(part 1 of 2)
# Autodesk Inventor assembly: Pins
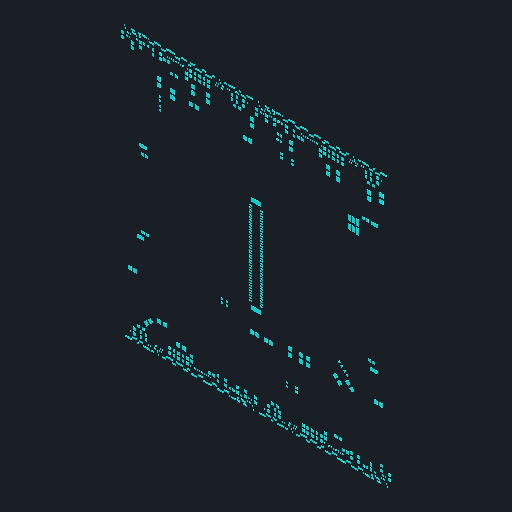
[picture p0: Inventor's stored thumbnail of the model, 512x512]
Saved by Autodesk Inventor 2027 (Build 310192060, 192F)
## iProperties
Created: 2026-07-14
Part Number: Pins
Description: PART--DESC
Document SubType Name: Assembly
Designer: caleb
Author: caleb
Revision Number: NONE
## Documents named in this file (559)
- C:\Users\caleb\Desktop\Shared\Software\Hardware\ETL\modules\Tamale v2.0\module_r50\Pins.iam
- C:\Users\caleb\Desktop\Shared\Software\Hardware\ETL\modules\Tamale v2.0\module_r50\1.ipt
- C:\Users\caleb\Desktop\Shared\Software\Hardware\ETL\modules\Tamale v2.0\module_r50\1_1.ipt
- C:\Users\caleb\Desktop\Shared\Software\Hardware\ETL\modules\Tamale v2.0\module_r50\1_2.ipt
- C:\Users\caleb\Desktop\Shared\Software\Hardware\ETL\modules\Tamale v2.0\module_r50\1_3.ipt
- C:\Users\caleb\Desktop\Shared\Software\Hardware\ETL\modules\Tamale v2.0\module_r50\1_4.ipt
- C:\Users\caleb\Desktop\Shared\Software\Hardware\ETL\modules\Tamale v2.0\module_r50\1_5.ipt
- C:\Users\caleb\Desktop\Shared\Software\Hardware\ETL\modules\Tamale v2.0\module_r50\1_6.ipt
- C:\Users\caleb\Desktop\Shared\Software\Hardware\ETL\modules\Tamale v2.0\module_r50\1_7.ipt
- C:\Users\caleb\Desktop\Shared\Software\Hardware\ETL\modules\Tamale v2.0\module_r50\1_8.ipt
- C:\Users\caleb\Desktop\Shared\Software\Hardware\ETL\modules\Tamale v2.0\module_r50\1_9.ipt
- C:\Users\caleb\Desktop\Shared\Software\Hardware\ETL\modules\Tamale v2.0\module_r50\1_10.ipt
- C:\Users\caleb\Desktop\Shared\Software\Hardware\ETL\modules\Tamale v2.0\module_r50\1_11.ipt
- C:\Users\caleb\Desktop\Shared\Software\Hardware\ETL\modules\Tamale v2.0\module_r50\1_12.ipt
- C:\Users\caleb\Desktop\Shared\Software\Hardware\ETL\modules\Tamale v2.0\module_r50\1_13.ipt
- C:\Users\caleb\Desktop\Shared\Software\Hardware\ETL\modules\Tamale v2.0\module_r50\1_14.ipt
- C:\Users\caleb\Desktop\Shared\Software\Hardware\ETL\modules\Tamale v2.0\module_r50\1_15.ipt
- C:\Users\caleb\Desktop\Shared\Software\Hardware\ETL\modules\Tamale v2.0\module_r50\1_16.ipt
- C:\Users\caleb\Desktop\Shared\Software\Hardware\ETL\modules\Tamale v2.0\module_r50\1_17.ipt
- C:\Users\caleb\Desktop\Shared\Software\Hardware\ETL\modules\Tamale v2.0\module_r50\1_18.ipt
- C:\Users\caleb\Desktop\Shared\Software\Hardware\ETL\modules\Tamale v2.0\module_r50\1_19.ipt
- C:\Users\caleb\Desktop\Shared\Software\Hardware\ETL\modules\Tamale v2.0\module_r50\1_20.ipt
- C:\Users\caleb\Desktop\Shared\Software\Hardware\ETL\modules\Tamale v2.0\module_r50\1_21.ipt
- C:\Users\caleb\Desktop\Shared\Software\Hardware\ETL\modules\Tamale v2.0\module_r50\1_22.ipt
- C:\Users\caleb\Desktop\Shared\Software\Hardware\ETL\modules\Tamale v2.0\module_r50\1_23.ipt
- C:\Users\caleb\Desktop\Shared\Software\Hardware\ETL\modules\Tamale v2.0\module_r50\1_24.ipt
- C:\Users\caleb\Desktop\Shared\Software\Hardware\ETL\modules\Tamale v2.0\module_r50\1_25.ipt
- C:\Users\caleb\Desktop\Shared\Software\Hardware\ETL\modules\Tamale v2.0\module_r50\1_26.ipt
- C:\Users\caleb\Desktop\Shared\Software\Hardware\ETL\modules\Tamale v2.0\module_r50\1_27.ipt
- C:\Users\caleb\Desktop\Shared\Software\Hardware\ETL\modules\Tamale v2.0\module_r50\1_28.ipt
- C:\Users\caleb\Desktop\Shared\Software\Hardware\ETL\modules\Tamale v2.0\module_r50\1_29.ipt
- C:\Users\caleb\Desktop\Shared\Software\Hardware\ETL\modules\Tamale v2.0\module_r50\1_30.ipt
- C:\Users\caleb\Desktop\Shared\Software\Hardware\ETL\modules\Tamale v2.0\module_r50\1_31.ipt
- C:\Users\caleb\Desktop\Shared\Software\Hardware\ETL\modules\Tamale v2.0\module_r50\1_32.ipt
- C:\Users\caleb\Desktop\Shared\Software\Hardware\ETL\modules\Tamale v2.0\module_r50\1_33.ipt
- C:\Users\caleb\Desktop\Shared\Software\Hardware\ETL\modules\Tamale v2.0\module_r50\1_34.ipt
- C:\Users\caleb\Desktop\Shared\Software\Hardware\ETL\modules\Tamale v2.0\module_r50\1_35.ipt
- C:\Users\caleb\Desktop\Shared\Software\Hardware\ETL\modules\Tamale v2.0\module_r50\1_36.ipt
- C:\Users\caleb\Desktop\Shared\Software\Hardware\ETL\modules\Tamale v2.0\module_r50\1_37.ipt
- C:\Users\caleb\Desktop\Shared\Software\Hardware\ETL\modules\Tamale v2.0\module_r50\1_38.ipt
- C:\Users\caleb\Desktop\Shared\Software\Hardware\ETL\modules\Tamale v2.0\module_r50\1_39.ipt
- C:\Users\caleb\Desktop\Shared\Software\Hardware\ETL\modules\Tamale v2.0\module_r50\1_40.ipt
- C:\Users\caleb\Desktop\Shared\Software\Hardware\ETL\modules\Tamale v2.0\module_r50\1_41.ipt
- C:\Users\caleb\Desktop\Shared\Software\Hardware\ETL\modules\Tamale v2.0\module_r50\1_42.ipt
- C:\Users\caleb\Desktop\Shared\Software\Hardware\ETL\modules\Tamale v2.0\module_r50\1_43.ipt
- C:\Users\caleb\Desktop\Shared\Software\Hardware\ETL\modules\Tamale v2.0\module_r50\1_44.ipt
- C:\Users\caleb\Desktop\Shared\Software\Hardware\ETL\modules\Tamale v2.0\module_r50\1_45.ipt
- C:\Users\caleb\Desktop\Shared\Software\Hardware\ETL\modules\Tamale v2.0\module_r50\1_46.ipt
- C:\Users\caleb\Desktop\Shared\Software\Hardware\ETL\modules\Tamale v2.0\module_r50\1_47.ipt
- C:\Users\caleb\Desktop\Shared\Software\Hardware\ETL\modules\Tamale v2.0\module_r50\1_48.ipt
- C:\Users\caleb\Desktop\Shared\Software\Hardware\ETL\modules\Tamale v2.0\module_r50\1_49.ipt
- C:\Users\caleb\Desktop\Shared\Software\Hardware\ETL\modules\Tamale v2.0\module_r50\1_50.ipt
- C:\Users\caleb\Desktop\Shared\Software\Hardware\ETL\modules\Tamale v2.0\module_r50\1_51.ipt
- C:\Users\caleb\Desktop\Shared\Software\Hardware\ETL\modules\Tamale v2.0\module_r50\1_52.ipt
- C:\Users\caleb\Desktop\Shared\Software\Hardware\ETL\modules\Tamale v2.0\module_r50\1_53.ipt
- C:\Users\caleb\Desktop\Shared\Software\Hardware\ETL\modules\Tamale v2.0\module_r50\1_54.ipt
- C:\Users\caleb\Desktop\Shared\Software\Hardware\ETL\modules\Tamale v2.0\module_r50\1_55.ipt
- C:\Users\caleb\Desktop\Shared\Software\Hardware\ETL\modules\Tamale v2.0\module_r50\1_56.ipt
- C:\Users\caleb\Desktop\Shared\Software\Hardware\ETL\modules\Tamale v2.0\module_r50\1_57.ipt
- C:\Users\caleb\Desktop\Shared\Software\Hardware\ETL\modules\Tamale v2.0\module_r50\1_58.ipt
- C:\Users\caleb\Desktop\Shared\Software\Hardware\ETL\modules\Tamale v2.0\module_r50\1_59.ipt
- C:\Users\caleb\Desktop\Shared\Software\Hardware\ETL\modules\Tamale v2.0\module_r50\1_60.ipt
- C:\Users\caleb\Desktop\Shared\Software\Hardware\ETL\modules\Tamale v2.0\module_r50\1_61.ipt
- C:\Users\caleb\Desktop\Shared\Software\Hardware\ETL\modules\Tamale v2.0\module_r50\1_62.ipt
- C:\Users\caleb\Desktop\Shared\Software\Hardware\ETL\modules\Tamale v2.0\module_r50\1_63.ipt
- C:\Users\caleb\Desktop\Shared\Software\Hardware\ETL\modules\Tamale v2.0\module_r50\1_64.ipt
- C:\Users\caleb\Desktop\Shared\Software\Hardware\ETL\modules\Tamale v2.0\module_r50\1_65.ipt
- C:\Users\caleb\Desktop\Shared\Software\Hardware\ETL\modules\Tamale v2.0\module_r50\1_66.ipt
- C:\Users\caleb\Desktop\Shared\Software\Hardware\ETL\modules\Tamale v2.0\module_r50\1_67.ipt
- C:\Users\caleb\Desktop\Shared\Software\Hardware\ETL\modules\Tamale v2.0\module_r50\1_68.ipt
- C:\Users\caleb\Desktop\Shared\Software\Hardware\ETL\modules\Tamale v2.0\module_r50\1_69.ipt
- C:\Users\caleb\Desktop\Shared\Software\Hardware\ETL\modules\Tamale v2.0\module_r50\1_70.ipt
- C:\Users\caleb\Desktop\Shared\Software\Hardware\ETL\modules\Tamale v2.0\module_r50\1_71.ipt
- C:\Users\caleb\Desktop\Shared\Software\Hardware\ETL\modules\Tamale v2.0\module_r50\1_72.ipt
- C:\Users\caleb\Desktop\Shared\Software\Hardware\ETL\modules\Tamale v2.0\module_r50\1_73.ipt
- C:\Users\caleb\Desktop\Shared\Software\Hardware\ETL\modules\Tamale v2.0\module_r50\1_74.ipt
- C:\Users\caleb\Desktop\Shared\Software\Hardware\ETL\modules\Tamale v2.0\module_r50\1_75.ipt
- C:\Users\caleb\Desktop\Shared\Software\Hardware\ETL\modules\Tamale v2.0\module_r50\1_76.ipt
- C:\Users\caleb\Desktop\Shared\Software\Hardware\ETL\modules\Tamale v2.0\module_r50\1_77.ipt
- C:\Users\caleb\Desktop\Shared\Software\Hardware\ETL\modules\Tamale v2.0\module_r50\1_78.ipt
- C:\Users\caleb\Desktop\Shared\Software\Hardware\ETL\modules\Tamale v2.0\module_r50\1_79.ipt
- C:\Users\caleb\Desktop\Shared\Software\Hardware\ETL\modules\Tamale v2.0\module_r50\1_80.ipt
- C:\Users\caleb\Desktop\Shared\Software\Hardware\ETL\modules\Tamale v2.0\module_r50\1_81.ipt
- C:\Users\caleb\Desktop\Shared\Software\Hardware\ETL\modules\Tamale v2.0\module_r50\1_82.ipt
- C:\Users\caleb\Desktop\Shared\Software\Hardware\ETL\modules\Tamale v2.0\module_r50\1_83.ipt
- C:\Users\caleb\Desktop\Shared\Software\Hardware\ETL\modules\Tamale v2.0\module_r50\1_84.ipt
- C:\Users\caleb\Desktop\Shared\Software\Hardware\ETL\modules\Tamale v2.0\module_r50\1_85.ipt
- C:\Users\caleb\Desktop\Shared\Software\Hardware\ETL\modules\Tamale v2.0\module_r50\1_86.ipt
- C:\Users\caleb\Desktop\Shared\Software\Hardware\ETL\modules\Tamale v2.0\module_r50\1_87.ipt
- C:\Users\caleb\Desktop\Shared\Software\Hardware\ETL\modules\Tamale v2.0\module_r50\1_88.ipt
- C:\Users\caleb\Desktop\Shared\Software\Hardware\ETL\modules\Tamale v2.0\module_r50\1_89.ipt
- C:\Users\caleb\Desktop\Shared\Software\Hardware\ETL\modules\Tamale v2.0\module_r50\1_90.ipt
- C:\Users\caleb\Desktop\Shared\Software\Hardware\ETL\modules\Tamale v2.0\module_r50\1_91.ipt
- C:\Users\caleb\Desktop\Shared\Software\Hardware\ETL\modules\Tamale v2.0\module_r50\1_92.ipt
- C:\Users\caleb\Desktop\Shared\Software\Hardware\ETL\modules\Tamale v2.0\module_r50\1_93.ipt
- C:\Users\caleb\Desktop\Shared\Software\Hardware\ETL\modules\Tamale v2.0\module_r50\1_94.ipt
- C:\Users\caleb\Desktop\Shared\Software\Hardware\ETL\modules\Tamale v2.0\module_r50\1_95.ipt
- C:\Users\caleb\Desktop\Shared\Software\Hardware\ETL\modules\Tamale v2.0\module_r50\1_96.ipt
- C:\Users\caleb\Desktop\Shared\Software\Hardware\ETL\modules\Tamale v2.0\module_r50\1_97.ipt
- C:\Users\caleb\Desktop\Shared\Software\Hardware\ETL\modules\Tamale v2.0\module_r50\1_98.ipt
- C:\Users\caleb\Desktop\Shared\Software\Hardware\ETL\modules\Tamale v2.0\module_r50\1_99.ipt
- C:\Users\caleb\Desktop\Shared\Software\Hardware\ETL\modules\Tamale v2.0\module_r50\1_100.ipt
- C:\Users\caleb\Desktop\Shared\Software\Hardware\ETL\modules\Tamale v2.0\module_r50\1_101.ipt
- C:\Users\caleb\Desktop\Shared\Software\Hardware\ETL\modules\Tamale v2.0\module_r50\1_102.ipt
- C:\Users\caleb\Desktop\Shared\Software\Hardware\ETL\modules\Tamale v2.0\module_r50\1_103.ipt
- C:\Users\caleb\Desktop\Shared\Software\Hardware\ETL\modules\Tamale v2.0\module_r50\1_104.ipt
- C:\Users\caleb\Desktop\Shared\Software\Hardware\ETL\modules\Tamale v2.0\module_r50\1_105.ipt
- C:\Users\caleb\Desktop\Shared\Software\Hardware\ETL\modules\Tamale v2.0\module_r50\1_106.ipt
- C:\Users\caleb\Desktop\Shared\Software\Hardware\ETL\modules\Tamale v2.0\module_r50\1_107.ipt
- C:\Users\caleb\Desktop\Shared\Software\Hardware\ETL\modules\Tamale v2.0\module_r50\1_108.ipt
- C:\Users\caleb\Desktop\Shared\Software\Hardware\ETL\modules\Tamale v2.0\module_r50\1_109.ipt
- C:\Users\caleb\Desktop\Shared\Software\Hardware\ETL\modules\Tamale v2.0\module_r50\1_110.ipt
- C:\Users\caleb\Desktop\Shared\Software\Hardware\ETL\modules\Tamale v2.0\module_r50\1_111.ipt
- C:\Users\caleb\Desktop\Shared\Software\Hardware\ETL\modules\Tamale v2.0\module_r50\1_112.ipt
- C:\Users\caleb\Desktop\Shared\Software\Hardware\ETL\modules\Tamale v2.0\module_r50\10.ipt
- C:\Users\caleb\Desktop\Shared\Software\Hardware\ETL\modules\Tamale v2.0\module_r50\11.ipt
- C:\Users\caleb\Desktop\Shared\Software\Hardware\ETL\modules\Tamale v2.0\module_r50\12.ipt
- C:\Users\caleb\Desktop\Shared\Software\Hardware\ETL\modules\Tamale v2.0\module_r50\13.ipt
- C:\Users\caleb\Desktop\Shared\Software\Hardware\ETL\modules\Tamale v2.0\module_r50\14.ipt
- C:\Users\caleb\Desktop\Shared\Software\Hardware\ETL\modules\Tamale v2.0\module_r50\15.ipt
- C:\Users\caleb\Desktop\Shared\Software\Hardware\ETL\modules\Tamale v2.0\module_r50\16.ipt
- C:\Users\caleb\Desktop\Shared\Software\Hardware\ETL\modules\Tamale v2.0\module_r50\17.ipt
- C:\Users\caleb\Desktop\Shared\Software\Hardware\ETL\modules\Tamale v2.0\module_r50\18.ipt
- C:\Users\caleb\Desktop\Shared\Software\Hardware\ETL\modules\Tamale v2.0\module_r50\19.ipt
- C:\Users\caleb\Desktop\Shared\Software\Hardware\ETL\modules\Tamale v2.0\module_r50\2.ipt
- C:\Users\caleb\Desktop\Shared\Software\Hardware\ETL\modules\Tamale v2.0\module_r50\2_1.ipt
- C:\Users\caleb\Desktop\Shared\Software\Hardware\ETL\modules\Tamale v2.0\module_r50\2_2.ipt
- C:\Users\caleb\Desktop\Shared\Software\Hardware\ETL\modules\Tamale v2.0\module_r50\2_3.ipt
- C:\Users\caleb\Desktop\Shared\Software\Hardware\ETL\modules\Tamale v2.0\module_r50\2_4.ipt
- C:\Users\caleb\Desktop\Shared\Software\Hardware\ETL\modules\Tamale v2.0\module_r50\2_5.ipt
- C:\Users\caleb\Desktop\Shared\Software\Hardware\ETL\modules\Tamale v2.0\module_r50\2_6.ipt
- C:\Users\caleb\Desktop\Shared\Software\Hardware\ETL\modules\Tamale v2.0\module_r50\2_7.ipt
- C:\Users\caleb\Desktop\Shared\Software\Hardware\ETL\modules\Tamale v2.0\module_r50\2_8.ipt
- C:\Users\caleb\Desktop\Shared\Software\Hardware\ETL\modules\Tamale v2.0\module_r50\2_9.ipt
- C:\Users\caleb\Desktop\Shared\Software\Hardware\ETL\modules\Tamale v2.0\module_r50\2_10.ipt
- C:\Users\caleb\Desktop\Shared\Software\Hardware\ETL\modules\Tamale v2.0\module_r50\2_11.ipt
- C:\Users\caleb\Desktop\Shared\Software\Hardware\ETL\modules\Tamale v2.0\module_r50\2_12.ipt
- C:\Users\caleb\Desktop\Shared\Software\Hardware\ETL\modules\Tamale v2.0\module_r50\2_13.ipt
- C:\Users\caleb\Desktop\Shared\Software\Hardware\ETL\modules\Tamale v2.0\module_r50\2_14.ipt
- C:\Users\caleb\Desktop\Shared\Software\Hardware\ETL\modules\Tamale v2.0\module_r50\2_15.ipt
- C:\Users\caleb\Desktop\Shared\Software\Hardware\ETL\modules\Tamale v2.0\module_r50\2_16.ipt
- C:\Users\caleb\Desktop\Shared\Software\Hardware\ETL\modules\Tamale v2.0\module_r50\2_17.ipt
- C:\Users\caleb\Desktop\Shared\Software\Hardware\ETL\modules\Tamale v2.0\module_r50\2_18.ipt
- C:\Users\caleb\Desktop\Shared\Software\Hardware\ETL\modules\Tamale v2.0\module_r50\2_19.ipt
- C:\Users\caleb\Desktop\Shared\Software\Hardware\ETL\modules\Tamale v2.0\module_r50\2_20.ipt
- C:\Users\caleb\Desktop\Shared\Software\Hardware\ETL\modules\Tamale v2.0\module_r50\2_21.ipt
- C:\Users\caleb\Desktop\Shared\Software\Hardware\ETL\modules\Tamale v2.0\module_r50\2_22.ipt
- C:\Users\caleb\Desktop\Shared\Software\Hardware\ETL\modules\Tamale v2.0\module_r50\2_23.ipt
- C:\Users\caleb\Desktop\Shared\Software\Hardware\ETL\modules\Tamale v2.0\module_r50\2_24.ipt
- C:\Users\caleb\Desktop\Shared\Software\Hardware\ETL\modules\Tamale v2.0\module_r50\2_25.ipt
- C:\Users\caleb\Desktop\Shared\Software\Hardware\ETL\modules\Tamale v2.0\module_r50\2_26.ipt
- C:\Users\caleb\Desktop\Shared\Software\Hardware\ETL\modules\Tamale v2.0\module_r50\2_27.ipt
- C:\Users\caleb\Desktop\Shared\Software\Hardware\ETL\modules\Tamale v2.0\module_r50\2_28.ipt
- C:\Users\caleb\Desktop\Shared\Software\Hardware\ETL\modules\Tamale v2.0\module_r50\2_29.ipt
- C:\Users\caleb\Desktop\Shared\Software\Hardware\ETL\modules\Tamale v2.0\module_r50\2_30.ipt
- C:\Users\caleb\Desktop\Shared\Software\Hardware\ETL\modules\Tamale v2.0\module_r50\2_31.ipt
- C:\Users\caleb\Desktop\Shared\Software\Hardware\ETL\modules\Tamale v2.0\module_r50\2_32.ipt
- C:\Users\caleb\Desktop\Shared\Software\Hardware\ETL\modules\Tamale v2.0\module_r50\2_33.ipt
- C:\Users\caleb\Desktop\Shared\Software\Hardware\ETL\modules\Tamale v2.0\module_r50\2_34.ipt
- C:\Users\caleb\Desktop\Shared\Software\Hardware\ETL\modules\Tamale v2.0\module_r50\2_35.ipt
- C:\Users\caleb\Desktop\Shared\Software\Hardware\ETL\modules\Tamale v2.0\module_r50\2_36.ipt
- C:\Users\caleb\Desktop\Shared\Software\Hardware\ETL\modules\Tamale v2.0\module_r50\2_37.ipt
- C:\Users\caleb\Desktop\Shared\Software\Hardware\ETL\modules\Tamale v2.0\module_r50\2_38.ipt
- C:\Users\caleb\Desktop\Shared\Software\Hardware\ETL\modules\Tamale v2.0\module_r50\2_39.ipt
- C:\Users\caleb\Desktop\Shared\Software\Hardware\ETL\modules\Tamale v2.0\module_r50\2_40.ipt
- C:\Users\caleb\Desktop\Shared\Software\Hardware\ETL\modules\Tamale v2.0\module_r50\2_41.ipt
- C:\Users\caleb\Desktop\Shared\Software\Hardware\ETL\modules\Tamale v2.0\module_r50\2_42.ipt
- C:\Users\caleb\Desktop\Shared\Software\Hardware\ETL\modules\Tamale v2.0\module_r50\2_43.ipt
- C:\Users\caleb\Desktop\Shared\Software\Hardware\ETL\modules\Tamale v2.0\module_r50\2_44.ipt
- C:\Users\caleb\Desktop\Shared\Software\Hardware\ETL\modules\Tamale v2.0\module_r50\2_45.ipt
- C:\Users\caleb\Desktop\Shared\Software\Hardware\ETL\modules\Tamale v2.0\module_r50\2_46.ipt
- C:\Users\caleb\Desktop\Shared\Software\Hardware\ETL\modules\Tamale v2.0\module_r50\2_47.ipt
- C:\Users\caleb\Desktop\Shared\Software\Hardware\ETL\modules\Tamale v2.0\module_r50\2_48.ipt
- C:\Users\caleb\Desktop\Shared\Software\Hardware\ETL\modules\Tamale v2.0\module_r50\2_49.ipt
- C:\Users\caleb\Desktop\Shared\Software\Hardware\ETL\modules\Tamale v2.0\module_r50\2_50.ipt
- C:\Users\caleb\Desktop\Shared\Software\Hardware\ETL\modules\Tamale v2.0\module_r50\2_51.ipt
- C:\Users\caleb\Desktop\Shared\Software\Hardware\ETL\modules\Tamale v2.0\module_r50\2_52.ipt
- C:\Users\caleb\Desktop\Shared\Software\Hardware\ETL\modules\Tamale v2.0\module_r50\2_53.ipt
- C:\Users\caleb\Desktop\Shared\Software\Hardware\ETL\modules\Tamale v2.0\module_r50\2_54.ipt
- C:\Users\caleb\Desktop\Shared\Software\Hardware\ETL\modules\Tamale v2.0\module_r50\2_55.ipt
- C:\Users\caleb\Desktop\Shared\Software\Hardware\ETL\modules\Tamale v2.0\module_r50\2_56.ipt
- C:\Users\caleb\Desktop\Shared\Software\Hardware\ETL\modules\Tamale v2.0\module_r50\2_57.ipt
- C:\Users\caleb\Desktop\Shared\Software\Hardware\ETL\modules\Tamale v2.0\module_r50\2_58.ipt
- C:\Users\caleb\Desktop\Shared\Software\Hardware\ETL\modules\Tamale v2.0\module_r50\2_59.ipt
- C:\Users\caleb\Desktop\Shared\Software\Hardware\ETL\modules\Tamale v2.0\module_r50\2_60.ipt
- C:\Users\caleb\Desktop\Shared\Software\Hardware\ETL\modules\Tamale v2.0\module_r50\2_61.ipt
- C:\Users\caleb\Desktop\Shared\Software\Hardware\ETL\modules\Tamale v2.0\module_r50\2_62.ipt
- C:\Users\caleb\Desktop\Shared\Software\Hardware\ETL\modules\Tamale v2.0\module_r50\2_63.ipt
- C:\Users\caleb\Desktop\Shared\Software\Hardware\ETL\modules\Tamale v2.0\module_r50\2_64.ipt
- C:\Users\caleb\Desktop\Shared\Software\Hardware\ETL\modules\Tamale v2.0\module_r50\2_65.ipt
- C:\Users\caleb\Desktop\Shared\Software\Hardware\ETL\modules\Tamale v2.0\module_r50\2_66.ipt
- C:\Users\caleb\Desktop\Shared\Software\Hardware\ETL\modules\Tamale v2.0\module_r50\2_67.ipt
- C:\Users\caleb\Desktop\Shared\Software\Hardware\ETL\modules\Tamale v2.0\module_r50\2_68.ipt
- C:\Users\caleb\Desktop\Shared\Software\Hardware\ETL\modules\Tamale v2.0\module_r50\2_69.ipt
- C:\Users\caleb\Desktop\Shared\Software\Hardware\ETL\modules\Tamale v2.0\module_r50\2_70.ipt
- C:\Users\caleb\Desktop\Shared\Software\Hardware\ETL\modules\Tamale v2.0\module_r50\2_71.ipt
- C:\Users\caleb\Desktop\Shared\Software\Hardware\ETL\modules\Tamale v2.0\module_r50\2_72.ipt
- C:\Users\caleb\Desktop\Shared\Software\Hardware\ETL\modules\Tamale v2.0\module_r50\2_73.ipt
- C:\Users\caleb\Desktop\Shared\Software\Hardware\ETL\modules\Tamale v2.0\module_r50\2_74.ipt
- C:\Users\caleb\Desktop\Shared\Software\Hardware\ETL\modules\Tamale v2.0\module_r50\2_75.ipt
- C:\Users\caleb\Desktop\Shared\Software\Hardware\ETL\modules\Tamale v2.0\module_r50\2_76.ipt
- C:\Users\caleb\Desktop\Shared\Software\Hardware\ETL\modules\Tamale v2.0\module_r50\2_77.ipt
- C:\Users\caleb\Desktop\Shared\Software\Hardware\ETL\modules\Tamale v2.0\module_r50\2_78.ipt
- C:\Users\caleb\Desktop\Shared\Software\Hardware\ETL\modules\Tamale v2.0\module_r50\2_79.ipt
- C:\Users\caleb\Desktop\Shared\Software\Hardware\ETL\modules\Tamale v2.0\module_r50\2_80.ipt
- C:\Users\caleb\Desktop\Shared\Software\Hardware\ETL\modules\Tamale v2.0\module_r50\2_81.ipt
- C:\Users\caleb\Desktop\Shared\Software\Hardware\ETL\modules\Tamale v2.0\module_r50\2_82.ipt
- C:\Users\caleb\Desktop\Shared\Software\Hardware\ETL\modules\Tamale v2.0\module_r50\2_83.ipt
- C:\Users\caleb\Desktop\Shared\Software\Hardware\ETL\modules\Tamale v2.0\module_r50\2_84.ipt
- C:\Users\caleb\Desktop\Shared\Software\Hardware\ETL\modules\Tamale v2.0\module_r50\2_85.ipt
- C:\Users\caleb\Desktop\Shared\Software\Hardware\ETL\modules\Tamale v2.0\module_r50\2_86.ipt
- C:\Users\caleb\Desktop\Shared\Software\Hardware\ETL\modules\Tamale v2.0\module_r50\2_87.ipt
- C:\Users\caleb\Desktop\Shared\Software\Hardware\ETL\modules\Tamale v2.0\module_r50\2_88.ipt
- C:\Users\caleb\Desktop\Shared\Software\Hardware\ETL\modules\Tamale v2.0\module_r50\2_89.ipt
- C:\Users\caleb\Desktop\Shared\Software\Hardware\ETL\modules\Tamale v2.0\module_r50\2_90.ipt
- C:\Users\caleb\Desktop\Shared\Software\Hardware\ETL\modules\Tamale v2.0\module_r50\2_91.ipt
- C:\Users\caleb\Desktop\Shared\Software\Hardware\ETL\modules\Tamale v2.0\module_r50\2_92.ipt
- C:\Users\caleb\Desktop\Shared\Software\Hardware\ETL\modules\Tamale v2.0\module_r50\2_93.ipt
- C:\Users\caleb\Desktop\Shared\Software\Hardware\ETL\modules\Tamale v2.0\module_r50\2_94.ipt
- C:\Users\caleb\Desktop\Shared\Software\Hardware\ETL\modules\Tamale v2.0\module_r50\2_95.ipt
- C:\Users\caleb\Desktop\Shared\Software\Hardware\ETL\modules\Tamale v2.0\module_r50\2_96.ipt
- C:\Users\caleb\Desktop\Shared\Software\Hardware\ETL\modules\Tamale v2.0\module_r50\2_97.ipt
- C:\Users\caleb\Desktop\Shared\Software\Hardware\ETL\modules\Tamale v2.0\module_r50\2_98.ipt
- C:\Users\caleb\Desktop\Shared\Software\Hardware\ETL\modules\Tamale v2.0\module_r50\2_99.ipt
- C:\Users\caleb\Desktop\Shared\Software\Hardware\ETL\modules\Tamale v2.0\module_r50\2_100.ipt
- C:\Users\caleb\Desktop\Shared\Software\Hardware\ETL\modules\Tamale v2.0\module_r50\2_101.ipt
- C:\Users\caleb\Desktop\Shared\Software\Hardware\ETL\modules\Tamale v2.0\module_r50\2_102.ipt
- C:\Users\caleb\Desktop\Shared\Software\Hardware\ETL\modules\Tamale v2.0\module_r50\2_103.ipt
- C:\Users\caleb\Desktop\Shared\Software\Hardware\ETL\modules\Tamale v2.0\module_r50\2_104.ipt
- C:\Users\caleb\Desktop\Shared\Software\Hardware\ETL\modules\Tamale v2.0\module_r50\2_105.ipt
- C:\Users\caleb\Desktop\Shared\Software\Hardware\ETL\modules\Tamale v2.0\module_r50\2_106.ipt
- C:\Users\caleb\Desktop\Shared\Software\Hardware\ETL\modules\Tamale v2.0\module_r50\2_107.ipt
- C:\Users\caleb\Desktop\Shared\Software\Hardware\ETL\modules\Tamale v2.0\module_r50\2_108.ipt
- C:\Users\caleb\Desktop\Shared\Software\Hardware\ETL\modules\Tamale v2.0\module_r50\2_109.ipt
- C:\Users\caleb\Desktop\Shared\Software\Hardware\ETL\modules\Tamale v2.0\module_r50\2_110.ipt
- C:\Users\caleb\Desktop\Shared\Software\Hardware\ETL\modules\Tamale v2.0\module_r50\2_111.ipt
- C:\Users\caleb\Desktop\Shared\Software\Hardware\ETL\modules\Tamale v2.0\module_r50\2_112.ipt
- C:\Users\caleb\Desktop\Shared\Software\Hardware\ETL\modules\Tamale v2.0\module_r50\20.ipt
- C:\Users\caleb\Desktop\Shared\Software\Hardware\ETL\modules\Tamale v2.0\module_r50\21.ipt
- C:\Users\caleb\Desktop\Shared\Software\Hardware\ETL\modules\Tamale v2.0\module_r50\22.ipt
- C:\Users\caleb\Desktop\Shared\Software\Hardware\ETL\modules\Tamale v2.0\module_r50\23.ipt
- C:\Users\caleb\Desktop\Shared\Software\Hardware\ETL\modules\Tamale v2.0\module_r50\24.ipt
- C:\Users\caleb\Desktop\Shared\Software\Hardware\ETL\modules\Tamale v2.0\module_r50\25.ipt
- C:\Users\caleb\Desktop\Shared\Software\Hardware\ETL\modules\Tamale v2.0\module_r50\26.ipt
- C:\Users\caleb\Desktop\Shared\Software\Hardware\ETL\modules\Tamale v2.0\module_r50\27.ipt
- C:\Users\caleb\Desktop\Shared\Software\Hardware\ETL\modules\Tamale v2.0\module_r50\28.ipt
- C:\Users\caleb\Desktop\Shared\Software\Hardware\ETL\modules\Tamale v2.0\module_r50\29.ipt
- C:\Users\caleb\Desktop\Shared\Software\Hardware\ETL\modules\Tamale v2.0\module_r50\3.ipt
- C:\Users\caleb\Desktop\Shared\Software\Hardware\ETL\modules\Tamale v2.0\module_r50\3_1.ipt
- C:\Users\caleb\Desktop\Shared\Software\Hardware\ETL\modules\Tamale v2.0\module_r50\3_2.ipt
- C:\Users\caleb\Desktop\Shared\Software\Hardware\ETL\modules\Tamale v2.0\module_r50\30.ipt
- C:\Users\caleb\Desktop\Shared\Software\Hardware\ETL\modules\Tamale v2.0\module_r50\31.ipt
- C:\Users\caleb\Desktop\Shared\Software\Hardware\ETL\modules\Tamale v2.0\module_r50\32.ipt
- C:\Users\caleb\Desktop\Shared\Software\Hardware\ETL\modules\Tamale v2.0\module_r50\33.ipt
- C:\Users\caleb\Desktop\Shared\Software\Hardware\ETL\modules\Tamale v2.0\module_r50\34.ipt
- C:\Users\caleb\Desktop\Shared\Software\Hardware\ETL\modules\Tamale v2.0\module_r50\35.ipt
- C:\Users\caleb\Desktop\Shared\Software\Hardware\ETL\modules\Tamale v2.0\module_r50\36.ipt
- C:\Users\caleb\Desktop\Shared\Software\Hardware\ETL\modules\Tamale v2.0\module_r50\37.ipt
- C:\Users\caleb\Desktop\Shared\Software\Hardware\ETL\modules\Tamale v2.0\module_r50\38.ipt
- C:\Users\caleb\Desktop\Shared\Software\Hardware\ETL\modules\Tamale v2.0\module_r50\39.ipt
- C:\Users\caleb\Desktop\Shared\Software\Hardware\ETL\modules\Tamale v2.0\module_r50\4.ipt
- C:\Users\caleb\Desktop\Shared\Software\Hardware\ETL\modules\Tamale v2.0\module_r50\40.ipt
- C:\Users\caleb\Desktop\Shared\Software\Hardware\ETL\modules\Tamale v2.0\module_r50\41.ipt
- C:\Users\caleb\Desktop\Shared\Software\Hardware\ETL\modules\Tamale v2.0\module_r50\42.ipt
- C:\Users\caleb\Desktop\Shared\Software\Hardware\ETL\modules\Tamale v2.0\module_r50\43.ipt
- C:\Users\caleb\Desktop\Shared\Software\Hardware\ETL\modules\Tamale v2.0\module_r50\44.ipt
- C:\Users\caleb\Desktop\Shared\Software\Hardware\ETL\modules\Tamale v2.0\module_r50\45.ipt
- C:\Users\caleb\Desktop\Shared\Software\Hardware\ETL\modules\Tamale v2.0\module_r50\46.ipt
- C:\Users\caleb\Desktop\Shared\Software\Hardware\ETL\modules\Tamale v2.0\module_r50\47.ipt
- C:\Users\caleb\Desktop\Shared\Software\Hardware\ETL\modules\Tamale v2.0\module_r50\48.ipt
- C:\Users\caleb\Desktop\Shared\Software\Hardware\ETL\modules\Tamale v2.0\module_r50\49.ipt
- C:\Users\caleb\Desktop\Shared\Software\Hardware\ETL\modules\Tamale v2.0\module_r50\5.ipt
- C:\Users\caleb\Desktop\Shared\Software\Hardware\ETL\modules\Tamale v2.0\module_r50\50.ipt
- C:\Users\caleb\Desktop\Shared\Software\Hardware\ETL\modules\Tamale v2.0\module_r50\51.ipt
- C:\Users\caleb\Desktop\Shared\Software\Hardware\ETL\modules\Tamale v2.0\module_r50\52.ipt
- C:\Users\caleb\Desktop\Shared\Software\Hardware\ETL\modules\Tamale v2.0\module_r50\53.ipt
- C:\Users\caleb\Desktop\Shared\Software\Hardware\ETL\modules\Tamale v2.0\module_r50\54.ipt
- C:\Users\caleb\Desktop\Shared\Software\Hardware\ETL\modules\Tamale v2.0\module_r50\55.ipt
- C:\Users\caleb\Desktop\Shared\Software\Hardware\ETL\modules\Tamale v2.0\module_r50\56.ipt
- C:\Users\caleb\Desktop\Shared\Software\Hardware\ETL\modules\Tamale v2.0\module_r50\57.ipt
- C:\Users\caleb\Desktop\Shared\Software\Hardware\ETL\modules\Tamale v2.0\module_r50\58.ipt
- C:\Users\caleb\Desktop\Shared\Software\Hardware\ETL\modules\Tamale v2.0\module_r50\59.ipt
- C:\Users\caleb\Desktop\Shared\Software\Hardware\ETL\modules\Tamale v2.0\module_r50\6.ipt
- C:\Users\caleb\Desktop\Shared\Software\Hardware\ETL\modules\Tamale v2.0\module_r50\60.ipt
- C:\Users\caleb\Desktop\Shared\Software\Hardware\ETL\modules\Tamale v2.0\module_r50\61.ipt
- C:\Users\caleb\Desktop\Shared\Software\Hardware\ETL\modules\Tamale v2.0\module_r50\62.ipt
- C:\Users\caleb\Desktop\Shared\Software\Hardware\ETL\modules\Tamale v2.0\module_r50\63.ipt
- C:\Users\caleb\Desktop\Shared\Software\Hardware\ETL\modules\Tamale v2.0\module_r50\64.ipt
- C:\Users\caleb\Desktop\Shared\Software\Hardware\ETL\modules\Tamale v2.0\module_r50\65.ipt
- C:\Users\caleb\Desktop\Shared\Software\Hardware\ETL\modules\Tamale v2.0\module_r50\66.ipt
- C:\Users\caleb\Desktop\Shared\Software\Hardware\ETL\modules\Tamale v2.0\module_r50\67.ipt
- C:\Users\caleb\Desktop\Shared\Software\Hardware\ETL\modules\Tamale v2.0\module_r50\68.ipt
- C:\Users\caleb\Desktop\Shared\Software\Hardware\ETL\modules\Tamale v2.0\module_r50\69.ipt
- C:\Users\caleb\Desktop\Shared\Software\Hardware\ETL\modules\Tamale v2.0\module_r50\7.ipt
- C:\Users\caleb\Desktop\Shared\Software\Hardware\ETL\modules\Tamale v2.0\module_r50\70.ipt
- C:\Users\caleb\Desktop\Shared\Software\Hardware\ETL\modules\Tamale v2.0\module_r50\71.ipt
- C:\Users\caleb\Desktop\Shared\Software\Hardware\ETL\modules\Tamale v2.0\module_r50\72.ipt
- C:\Users\caleb\Desktop\Shared\Software\Hardware\ETL\modules\Tamale v2.0\module_r50\73.ipt
- C:\Users\caleb\Desktop\Shared\Software\Hardware\ETL\modules\Tamale v2.0\module_r50\74.ipt
- C:\Users\caleb\Desktop\Shared\Software\Hardware\ETL\modules\Tamale v2.0\module_r50\75.ipt
- C:\Users\caleb\Desktop\Shared\Software\Hardware\ETL\modules\Tamale v2.0\module_r50\76.ipt
- C:\Users\caleb\Desktop\Shared\Software\Hardware\ETL\modules\Tamale v2.0\module_r50\77.ipt
- C:\Users\caleb\Desktop\Shared\Software\Hardware\ETL\modules\Tamale v2.0\module_r50\78.ipt
- C:\Users\caleb\Desktop\Shared\Software\Hardware\ETL\modules\Tamale v2.0\module_r50\8.ipt
- C:\Users\caleb\Desktop\Shared\Software\Hardware\ETL\modules\Tamale v2.0\module_r50\9.ipt
- C:\Users\caleb\Desktop\Shared\Software\Hardware\ETL\modules\Tamale v2.0\module_r50\CLK1280_N.ipt
- C:\Users\caleb\Desktop\Shared\Software\Hardware\ETL\modules\Tamale v2.0\module_r50\CLK1280_N_1.ipt
- C:\Users\caleb\Desktop\Shared\Software\Hardware\ETL\modules\Tamale v2.0\module_r50\CLK1280_N_2.ipt
- C:\Users\caleb\Desktop\Shared\Software\Hardware\ETL\modules\Tamale v2.0\module_r50\CLK1280_N_3.ipt
- C:\Users\caleb\Desktop\Shared\Software\Hardware\ETL\modules\Tamale v2.0\module_r50\CLK1280_P.ipt
- C:\Users\caleb\Desktop\Shared\Software\Hardware\ETL\modules\Tamale v2.0\module_r50\CLK1280_P_1.ipt
- C:\Users\caleb\Desktop\Shared\Software\Hardware\ETL\modules\Tamale v2.0\module_r50\CLK1280_P_2.ipt
- C:\Users\caleb\Desktop\Shared\Software\Hardware\ETL\modules\Tamale v2.0\module_r50\CLK1280_P_3.ipt
- C:\Users\caleb\Desktop\Shared\Software\Hardware\ETL\modules\Tamale v2.0\module_r50\CLK40_N.ipt
- C:\Users\caleb\Desktop\Shared\Software\Hardware\ETL\modules\Tamale v2.0\module_r50\CLK40_N_1.ipt
- C:\Users\caleb\Desktop\Shared\Software\Hardware\ETL\modules\Tamale v2.0\module_r50\CLK40_N_2.ipt
- C:\Users\caleb\Desktop\Shared\Software\Hardware\ETL\modules\Tamale v2.0\module_r50\CLK40_N_3.ipt
- C:\Users\caleb\Desktop\Shared\Software\Hardware\ETL\modules\Tamale v2.0\module_r50\CLK40_P.ipt
- C:\Users\caleb\Desktop\Shared\Software\Hardware\ETL\modules\Tamale v2.0\module_r50\CLK40_P_1.ipt
- C:\Users\caleb\Desktop\Shared\Software\Hardware\ETL\modules\Tamale v2.0\module_r50\CLK40_P_2.ipt
- C:\Users\caleb\Desktop\Shared\Software\Hardware\ETL\modules\Tamale v2.0\module_r50\CLK40_P_3.ipt
- C:\Users\caleb\Desktop\Shared\Software\Hardware\ETL\modules\Tamale v2.0\module_r50\DOL_N.ipt
- C:\Users\caleb\Desktop\Shared\Software\Hardware\ETL\modules\Tamale v2.0\module_r50\DOL_N_1.ipt
- C:\Users\caleb\Desktop\Shared\Software\Hardware\ETL\modules\Tamale v2.0\module_r50\DOL_N_2.ipt
- C:\Users\caleb\Desktop\Shared\Software\Hardware\ETL\modules\Tamale v2.0\module_r50\DOL_N_3.ipt
- C:\Users\caleb\Desktop\Shared\Software\Hardware\ETL\modules\Tamale v2.0\module_r50\DOL_P.ipt
- C:\Users\caleb\Desktop\Shared\Software\Hardware\ETL\modules\Tamale v2.0\module_r50\DOL_P_1.ipt
- C:\Users\caleb\Desktop\Shared\Software\Hardware\ETL\modules\Tamale v2.0\module_r50\DOL_P_2.ipt
- C:\Users\caleb\Desktop\Shared\Software\Hardware\ETL\modules\Tamale v2.0\module_r50\DOL_P_3.ipt
- C:\Users\caleb\Desktop\Shared\Software\Hardware\ETL\modules\Tamale v2.0\module_r50\DOR_N.ipt
- C:\Users\caleb\Desktop\Shared\Software\Hardware\ETL\modules\Tamale v2.0\module_r50\DOR_N_1.ipt
- C:\Users\caleb\Desktop\Shared\Software\Hardware\ETL\modules\Tamale v2.0\module_r50\DOR_N_2.ipt
- C:\Users\caleb\Desktop\Shared\Software\Hardware\ETL\modules\Tamale v2.0\module_r50\DOR_N_3.ipt
- C:\Users\caleb\Desktop\Shared\Software\Hardware\ETL\modules\Tamale v2.0\module_r50\DOR_P.ipt
- C:\Users\caleb\Desktop\Shared\Software\Hardware\ETL\modules\Tamale v2.0\module_r50\DOR_P_1.ipt
- C:\Users\caleb\Desktop\Shared\Software\Hardware\ETL\modules\Tamale v2.0\module_r50\DOR_P_2.ipt
- C:\Users\caleb\Desktop\Shared\Software\Hardware\ETL\modules\Tamale v2.0\module_r50\DOR_P_3.ipt
- C:\Users\caleb\Desktop\Shared\Software\Hardware\ETL\modules\Tamale v2.0\module_r50\FCN.ipt
- C:\Users\caleb\Desktop\Shared\Software\Hardware\ETL\modules\Tamale v2.0\module_r50\FCN_1.ipt
- C:\Users\caleb\Desktop\Shared\Software\Hardware\ETL\modules\Tamale v2.0\module_r50\FCN_2.ipt
- C:\Users\caleb\Desktop\Shared\Software\Hardware\ETL\modules\Tamale v2.0\module_r50\FCN_3.ipt
- C:\Users\caleb\Desktop\Shared\Software\Hardware\ETL\modules\Tamale v2.0\module_r50\FCP.ipt
- C:\Users\caleb\Desktop\Shared\Software\Hardware\ETL\modules\Tamale v2.0\module_r50\FCP_1.ipt
- C:\Users\caleb\Desktop\Shared\Software\Hardware\ETL\modules\Tamale v2.0\module_r50\FCP_2.ipt
- C:\Users\caleb\Desktop\Shared\Software\Hardware\ETL\modules\Tamale v2.0\module_r50\FCP_3.ipt
- C:\Users\caleb\Desktop\Shared\Software\Hardware\ETL\modules\Tamale v2.0\module_r50\I2C_ADDR0.ipt
- C:\Users\caleb\Desktop\Shared\Software\Hardware\ETL\modules\Tamale v2.0\module_r50\I2C_ADDR0_1.ipt
- C:\Users\caleb\Desktop\Shared\Software\Hardware\ETL\modules\Tamale v2.0\module_r50\I2C_ADDR0_2.ipt
- C:\Users\caleb\Desktop\Shared\Software\Hardware\ETL\modules\Tamale v2.0\module_r50\I2C_ADDR0_3.ipt
- C:\Users\caleb\Desktop\Shared\Software\Hardware\ETL\modules\Tamale v2.0\module_r50\I2C_ADDR1.ipt
- C:\Users\caleb\Desktop\Shared\Software\Hardware\ETL\modules\Tamale v2.0\module_r50\I2C_ADDR1_1.ipt
- C:\Users\caleb\Desktop\Shared\Software\Hardware\ETL\modules\Tamale v2.0\module_r50\I2C_ADDR1_2.ipt
- C:\Users\caleb\Desktop\Shared\Software\Hardware\ETL\modules\Tamale v2.0\module_r50\I2C_ADDR1_3.ipt
- C:\Users\caleb\Desktop\Shared\Software\Hardware\ETL\modules\Tamale v2.0\module_r50\I2C_ADDR2.ipt
- C:\Users\caleb\Desktop\Shared\Software\Hardware\ETL\modules\Tamale v2.0\module_r50\I2C_ADDR2_1.ipt
- C:\Users\caleb\Desktop\Shared\Software\Hardware\ETL\modules\Tamale v2.0\module_r50\I2C_ADDR2_2.ipt
- C:\Users\caleb\Desktop\Shared\Software\Hardware\ETL\modules\Tamale v2.0\module_r50\I2C_ADDR2_3.ipt
- C:\Users\caleb\Desktop\Shared\Software\Hardware\ETL\modules\Tamale v2.0\module_r50\I2C_ADDR3.ipt
- C:\Users\caleb\Desktop\Shared\Software\Hardware\ETL\modules\Tamale v2.0\module_r50\I2C_ADDR3_1.ipt
- C:\Users\caleb\Desktop\Shared\Software\Hardware\ETL\modules\Tamale v2.0\module_r50\I2C_ADDR3_2.ipt
- C:\Users\caleb\Desktop\Shared\Software\Hardware\ETL\modules\Tamale v2.0\module_r50\I2C_ADDR3_3.ipt
- C:\Users\caleb\Desktop\Shared\Software\Hardware\ETL\modules\Tamale v2.0\module_r50\I2C_ADDR4.ipt
- C:\Users\caleb\Desktop\Shared\Software\Hardware\ETL\modules\Tamale v2.0\module_r50\I2C_ADDR4_1.ipt
- C:\Users\caleb\Desktop\Shared\Software\Hardware\ETL\modules\Tamale v2.0\module_r50\I2C_ADDR4_2.ipt
- C:\Users\caleb\Desktop\Shared\Software\Hardware\ETL\modules\Tamale v2.0\module_r50\I2C_ADDR4_3.ipt
- C:\Users\caleb\Desktop\Shared\Software\Hardware\ETL\modules\Tamale v2.0\module_r50\POWER1.ipt
- C:\Users\caleb\Desktop\Shared\Software\Hardware\ETL\modules\Tamale v2.0\module_r50\POWER2.ipt
- C:\Users\caleb\Desktop\Shared\Software\Hardware\ETL\modules\Tamale v2.0\module_r50\RSTN.ipt
- C:\Users\caleb\Desktop\Shared\Software\Hardware\ETL\modules\Tamale v2.0\module_r50\RSTN_1.ipt
- C:\Users\caleb\Desktop\Shared\Software\Hardware\ETL\modules\Tamale v2.0\module_r50\RSTN_2.ipt
- C:\Users\caleb\Desktop\Shared\Software\Hardware\ETL\modules\Tamale v2.0\module_r50\RSTN_3.ipt
- C:\Users\caleb\Desktop\Shared\Software\Hardware\ETL\modules\Tamale v2.0\module_r50\SCL.ipt
- C:\Users\caleb\Desktop\Shared\Software\Hardware\ETL\modules\Tamale v2.0\module_r50\SCL_1.ipt
- C:\Users\caleb\Desktop\Shared\Software\Hardware\ETL\modules\Tamale v2.0\module_r50\SCL_2.ipt
- C:\Users\caleb\Desktop\Shared\Software\Hardware\ETL\modules\Tamale v2.0\module_r50\SCL_3.ipt
- C:\Users\caleb\Desktop\Shared\Software\Hardware\ETL\modules\Tamale v2.0\module_r50\SDA.ipt
- C:\Users\caleb\Desktop\Shared\Software\Hardware\ETL\modules\Tamale v2.0\module_r50\SDA_1.ipt
- C:\Users\caleb\Desktop\Shared\Software\Hardware\ETL\modules\Tamale v2.0\module_r50\SDA_2.ipt
- C:\Users\caleb\Desktop\Shared\Software\Hardware\ETL\modules\Tamale v2.0\module_r50\SDA_3.ipt
- C:\Users\caleb\Desktop\Shared\Software\Hardware\ETL\modules\Tamale v2.0\module_r50\TP.ipt
- C:\Users\caleb\Desktop\Shared\Software\Hardware\ETL\modules\Tamale v2.0\module_r50\TP_1.ipt
- C:\Users\caleb\Desktop\Shared\Software\Hardware\ETL\modules\Tamale v2.0\module_r50\TP_2.ipt
- C:\Users\caleb\Desktop\Shared\Software\Hardware\ETL\modules\Tamale v2.0\module_r50\TP_3.ipt
- C:\Users\caleb\Desktop\Shared\Software\Hardware\ETL\modules\Tamale v2.0\module_r50\VDD_A.ipt
- C:\Users\caleb\Desktop\Shared\Software\Hardware\ETL\modules\Tamale v2.0\module_r50\VDD_A_1.ipt
- C:\Users\caleb\Desktop\Shared\Software\Hardware\ETL\modules\Tamale v2.0\module_r50\VDD_A_2.ipt
- C:\Users\caleb\Desktop\Shared\Software\Hardware\ETL\modules\Tamale v2.0\module_r50\VDD_A_3.ipt
- C:\Users\caleb\Desktop\Shared\Software\Hardware\ETL\modules\Tamale v2.0\module_r50\VDD_A1.ipt
- C:\Users\caleb\Desktop\Shared\Software\Hardware\ETL\modules\Tamale v2.0\module_r50\VDD_A1_1.ipt
- C:\Users\caleb\Desktop\Shared\Software\Hardware\ETL\modules\Tamale v2.0\module_r50\VDD_A1_2.ipt
- C:\Users\caleb\Desktop\Shared\Software\Hardware\ETL\modules\Tamale v2.0\module_r50\VDD_A1_3.ipt
- C:\Users\caleb\Desktop\Shared\Software\Hardware\ETL\modules\Tamale v2.0\module_r50\VDD_A12.ipt
- C:\Users\caleb\Desktop\Shared\Software\Hardware\ETL\modules\Tamale v2.0\module_r50\VDD_A12_1.ipt
- C:\Users\caleb\Desktop\Shared\Software\Hardware\ETL\modules\Tamale v2.0\module_r50\VDD_A12_2.ipt
- C:\Users\caleb\Desktop\Shared\Software\Hardware\ETL\modules\Tamale v2.0\module_r50\VDD_A12_3.ipt
- C:\Users\caleb\Desktop\Shared\Software\Hardware\ETL\modules\Tamale v2.0\module_r50\VDD_A5.ipt
- C:\Users\caleb\Desktop\Shared\Software\Hardware\ETL\modules\Tamale v2.0\module_r50\VDD_A5_1.ipt
- C:\Users\caleb\Desktop\Shared\Software\Hardware\ETL\modules\Tamale v2.0\module_r50\VDD_A5_2.ipt
- C:\Users\caleb\Desktop\Shared\Software\Hardware\ETL\modules\Tamale v2.0\module_r50\VDD_A5_3.ipt
- C:\Users\caleb\Desktop\Shared\Software\Hardware\ETL\modules\Tamale v2.0\module_r50\VDD_D.ipt
- C:\Users\caleb\Desktop\Shared\Software\Hardware\ETL\modules\Tamale v2.0\module_r50\VDD_D_1.ipt
- C:\Users\caleb\Desktop\Shared\Software\Hardware\ETL\modules\Tamale v2.0\module_r50\VDD_D_2.ipt
- C:\Users\caleb\Desktop\Shared\Software\Hardware\ETL\modules\Tamale v2.0\module_r50\VDD_D_3.ipt
- C:\Users\caleb\Desktop\Shared\Software\Hardware\ETL\modules\Tamale v2.0\module_r50\VDD_D11.ipt
- C:\Users\caleb\Desktop\Shared\Software\Hardware\ETL\modules\Tamale v2.0\module_r50\VDD_D11_1.ipt
- C:\Users\caleb\Desktop\Shared\Software\Hardware\ETL\modules\Tamale v2.0\module_r50\VDD_D11_2.ipt
- C:\Users\caleb\Desktop\Shared\Software\Hardware\ETL\modules\Tamale v2.0\module_r50\VDD_D11_3.ipt
- C:\Users\caleb\Desktop\Shared\Software\Hardware\ETL\modules\Tamale v2.0\module_r50\VDD_D15.ipt
- C:\Users\caleb\Desktop\Shared\Software\Hardware\ETL\modules\Tamale v2.0\module_r50\VDD_D15_1.ipt
- C:\Users\caleb\Desktop\Shared\Software\Hardware\ETL\modules\Tamale v2.0\module_r50\VDD_D15_2.ipt
- C:\Users\caleb\Desktop\Shared\Software\Hardware\ETL\modules\Tamale v2.0\module_r50\VDD_D15_3.ipt
- C:\Users\caleb\Desktop\Shared\Software\Hardware\ETL\modules\Tamale v2.0\module_r50\VDD_D20.ipt
- C:\Users\caleb\Desktop\Shared\Software\Hardware\ETL\modules\Tamale v2.0\module_r50\VDD_D20_1.ipt
- C:\Users\caleb\Desktop\Shared\Software\Hardware\ETL\modules\Tamale v2.0\module_r50\VDD_D20_2.ipt
- C:\Users\caleb\Desktop\Shared\Software\Hardware\ETL\modules\Tamale v2.0\module_r50\VDD_D20_3.ipt
- C:\Users\caleb\Desktop\Shared\Software\Hardware\ETL\modules\Tamale v2.0\module_r50\VDD_D21.ipt
- C:\Users\caleb\Desktop\Shared\Software\Hardware\ETL\modules\Tamale v2.0\module_r50\VDD_D21_1.ipt
- C:\Users\caleb\Desktop\Shared\Software\Hardware\ETL\modules\Tamale v2.0\module_r50\VDD_D21_2.ipt
- C:\Users\caleb\Desktop\Shared\Software\Hardware\ETL\modules\Tamale v2.0\module_r50\VDD_D21_3.ipt
- C:\Users\caleb\Desktop\Shared\Software\Hardware\ETL\modules\Tamale v2.0\module_r50\VDD_EFUSE.ipt
- C:\Users\caleb\Desktop\Shared\Software\Hardware\ETL\modules\Tamale v2.0\module_r50\VDD_EFUSE_1.ipt
- C:\Users\caleb\Desktop\Shared\Software\Hardware\ETL\modules\Tamale v2.0\module_r50\VDD_EFUSE_2.ipt
- C:\Users\caleb\Desktop\Shared\Software\Hardware\ETL\modules\Tamale v2.0\module_r50\VDD_EFUSE_3.ipt
- C:\Users\caleb\Desktop\Shared\Software\Hardware\ETL\modules\Tamale v2.0\module_r50\VP.ipt
- C:\Users\caleb\Desktop\Shared\Software\Hardware\ETL\modules\Tamale v2.0\module_r50\VP_1.ipt
- C:\Users\caleb\Desktop\Shared\Software\Hardware\ETL\modules\Tamale v2.0\module_r50\VP_2.ipt
- C:\Users\caleb\Desktop\Shared\Software\Hardware\ETL\modules\Tamale v2.0\module_r50\VP_3.ipt
- C:\Users\caleb\Desktop\Shared\Software\Hardware\ETL\modules\Tamale v2.0\module_r50\VREF.ipt
- C:\Users\caleb\Desktop\Shared\Software\Hardware\ETL\modules\Tamale v2.0\module_r50\VREF_1.ipt
- C:\Users\caleb\Desktop\Shared\Software\Hardware\ETL\modules\Tamale v2.0\module_r50\VREF_2.ipt
- C:\Users\caleb\Desktop\Shared\Software\Hardware\ETL\modules\Tamale v2.0\module_r50\VREF_3.ipt
- C:\Users\caleb\Desktop\Shared\Software\Hardware\ETL\modules\Tamale v2.0\module_r50\VSS_A.ipt
- C:\Users\caleb\Desktop\Shared\Software\Hardware\ETL\modules\Tamale v2.0\module_r50\VSS_A_1.ipt
- C:\Users\caleb\Desktop\Shared\Software\Hardware\ETL\modules\Tamale v2.0\module_r50\VSS_A_2.ipt
- C:\Users\caleb\Desktop\Shared\Software\Hardware\ETL\modules\Tamale v2.0\module_r50\VSS_A_3.ipt
- C:\Users\caleb\Desktop\Shared\Software\Hardware\ETL\modules\Tamale v2.0\module_r50\VSS_A2.ipt
- C:\Users\caleb\Desktop\Shared\Software\Hardware\ETL\modules\Tamale v2.0\module_r50\VSS_A2_1.ipt
- C:\Users\caleb\Desktop\Shared\Software\Hardware\ETL\modules\Tamale v2.0\module_r50\VSS_A2_2.ipt
- C:\Users\caleb\Desktop\Shared\Software\Hardware\ETL\modules\Tamale v2.0\module_r50\VSS_A2_3.ipt
- C:\Users\caleb\Desktop\Shared\Software\Hardware\ETL\modules\Tamale v2.0\module_r50\VSS_A22.ipt
- C:\Users\caleb\Desktop\Shared\Software\Hardware\ETL\modules\Tamale v2.0\module_r50\VSS_A22_1.ipt
- C:\Users\caleb\Desktop\Shared\Software\Hardware\ETL\modules\Tamale v2.0\module_r50\VSS_A22_2.ipt
- C:\Users\caleb\Desktop\Shared\Software\Hardware\ETL\modules\Tamale v2.0\module_r50\VSS_A22_3.ipt
- C:\Users\caleb\Desktop\Shared\Software\Hardware\ETL\modules\Tamale v2.0\module_r50\VSS_A3.ipt
- C:\Users\caleb\Desktop\Shared\Software\Hardware\ETL\modules\Tamale v2.0\module_r50\VSS_A3_1.ipt
- C:\Users\caleb\Desktop\Shared\Software\Hardware\ETL\modules\Tamale v2.0\module_r50\VSS_A3_2.ipt
- C:\Users\caleb\Desktop\Shared\Software\Hardware\ETL\modules\Tamale v2.0\module_r50\VSS_A3_3.ipt
- C:\Users\caleb\Desktop\Shared\Software\Hardware\ETL\modules\Tamale v2.0\module_r50\VSS_A4.ipt
- C:\Users\caleb\Desktop\Shared\Software\Hardware\ETL\modules\Tamale v2.0\module_r50\VSS_A4_1.ipt
- C:\Users\caleb\Desktop\Shared\Software\Hardware\ETL\modules\Tamale v2.0\module_r50\VSS_A4_2.ipt
- C:\Users\caleb\Desktop\Shared\Software\Hardware\ETL\modules\Tamale v2.0\module_r50\VSS_A4_3.ipt
- C:\Users\caleb\Desktop\Shared\Software\Hardware\ETL\modules\Tamale v2.0\module_r50\VSS_A9.ipt
- C:\Users\caleb\Desktop\Shared\Software\Hardware\ETL\modules\Tamale v2.0\module_r50\VSS_A9_1.ipt
- C:\Users\caleb\Desktop\Shared\Software\Hardware\ETL\modules\Tamale v2.0\module_r50\VSS_A9_2.ipt
- C:\Users\caleb\Desktop\Shared\Software\Hardware\ETL\modules\Tamale v2.0\module_r50\VSS_A9_3.ipt
- C:\Users\caleb\Desktop\Shared\Software\Hardware\ETL\modules\Tamale v2.0\module_r50\VSS_AO.ipt
- C:\Users\caleb\Desktop\Shared\Software\Hardware\ETL\modules\Tamale v2.0\module_r50\VSS_AO_1.ipt
- C:\Users\caleb\Desktop\Shared\Software\Hardware\ETL\modules\Tamale v2.0\module_r50\VSS_AO_2.ipt
- C:\Users\caleb\Desktop\Shared\Software\Hardware\ETL\modules\Tamale v2.0\module_r50\VSS_AO_3.ipt
- C:\Users\caleb\Desktop\Shared\Software\Hardware\ETL\modules\Tamale v2.0\module_r50\VSS_D.ipt
- C:\Users\caleb\Desktop\Shared\Software\Hardware\ETL\modules\Tamale v2.0\module_r50\VSS_D_1.ipt
- C:\Users\caleb\Desktop\Shared\Software\Hardware\ETL\modules\Tamale v2.0\module_r50\VSS_D_2.ipt
- C:\Users\caleb\Desktop\Shared\Software\Hardware\ETL\modules\Tamale v2.0\module_r50\VSS_D_3.ipt
- C:\Users\caleb\Desktop\Shared\Software\Hardware\ETL\modules\Tamale v2.0\module_r50\VSS_D13.ipt
- C:\Users\caleb\Desktop\Shared\Software\Hardware\ETL\modules\Tamale v2.0\module_r50\VSS_D13_1.ipt
- C:\Users\caleb\Desktop\Shared\Software\Hardware\ETL\modules\Tamale v2.0\module_r50\VSS_D13_2.ipt
- C:\Users\caleb\Desktop\Shared\Software\Hardware\ETL\modules\Tamale v2.0\module_r50\VSS_D13_3.ipt
- C:\Users\caleb\Desktop\Shared\Software\Hardware\ETL\modules\Tamale v2.0\module_r50\VSS_D14.ipt
- C:\Users\caleb\Desktop\Shared\Software\Hardware\ETL\modules\Tamale v2.0\module_r50\VSS_D14_1.ipt
- C:\Users\caleb\Desktop\Shared\Software\Hardware\ETL\modules\Tamale v2.0\module_r50\VSS_D14_2.ipt
- C:\Users\caleb\Desktop\Shared\Software\Hardware\ETL\modules\Tamale v2.0\module_r50\VSS_D14_3.ipt
- C:\Users\caleb\Desktop\Shared\Software\Hardware\ETL\modules\Tamale v2.0\module_r50\VSS_D16.ipt
- C:\Users\caleb\Desktop\Shared\Software\Hardware\ETL\modules\Tamale v2.0\module_r50\VSS_D16_1.ipt
- C:\Users\caleb\Desktop\Shared\Software\Hardware\ETL\modules\Tamale v2.0\module_r50\VSS_D16_2.ipt
- C:\Users\caleb\Desktop\Shared\Software\Hardware\ETL\modules\Tamale v2.0\module_r50\VSS_D16_3.ipt
- C:\Users\caleb\Desktop\Shared\Software\Hardware\ETL\modules\Tamale v2.0\module_r50\VSS_D17.ipt
- C:\Users\caleb\Desktop\Shared\Software\Hardware\ETL\modules\Tamale v2.0\module_r50\VSS_D17_1.ipt
- C:\Users\caleb\Desktop\Shared\Software\Hardware\ETL\modules\Tamale v2.0\module_r50\VSS_D17_2.ipt
- C:\Users\caleb\Desktop\Shared\Software\Hardware\ETL\modules\Tamale v2.0\module_r50\VSS_D17_3.ipt
- C:\Users\caleb\Desktop\Shared\Software\Hardware\ETL\modules\Tamale v2.0\module_r50\VSS_D18.ipt
- C:\Users\caleb\Desktop\Shared\Software\Hardware\ETL\modules\Tamale v2.0\module_r50\VSS_D18_1.ipt
- C:\Users\caleb\Desktop\Shared\Software\Hardware\ETL\modules\Tamale v2.0\module_r50\VSS_D18_2.ipt
- C:\Users\caleb\Desktop\Shared\Software\Hardware\ETL\modules\Tamale v2.0\module_r50\VSS_D18_3.ipt
- C:\Users\caleb\Desktop\Shared\Software\Hardware\ETL\modules\Tamale v2.0\module_r50\VSS_D19.ipt
- C:\Users\caleb\Desktop\Shared\Software\Hardware\ETL\modules\Tamale v2.0\module_r50\VSS_D19_1.ipt
- C:\Users\caleb\Desktop\Shared\Software\Hardware\ETL\modules\Tamale v2.0\module_r50\VSS_D19_2.ipt
- C:\Users\caleb\Desktop\Shared\Software\Hardware\ETL\modules\Tamale v2.0\module_r50\VSS_D19_3.ipt
- C:\Users\caleb\Desktop\Shared\Software\Hardware\ETL\modules\Tamale v2.0\module_r50\VTEMP.ipt
- C:\Users\caleb\Desktop\Shared\Software\Hardware\ETL\modules\Tamale v2.0\module_r50\VTEMP_1.ipt
- C:\Users\caleb\Desktop\Shared\Software\Hardware\ETL\modules\Tamale v2.0\module_r50\VTEMP_2.ipt
- C:\Users\caleb\Desktop\Shared\Software\Hardware\ETL\modules\Tamale v2.0\module_r50\VTEMP_3.ipt
- C:\Users\caleb\Desktop\Shared\Software\Hardware\ETL\modules\Tamale v2.0\module_r50\WS_ADDR0.ipt
- C:\Users\caleb\Desktop\Shared\Software\Hardware\ETL\modules\Tamale v2.0\module_r50\WS_ADDR0_1.ipt
- C:\Users\caleb\Desktop\Shared\Software\Hardware\ETL\modules\Tamale v2.0\module_r50\WS_ADDR0_2.ipt
- C:\Users\caleb\Desktop\Shared\Software\Hardware\ETL\modules\Tamale v2.0\module_r50\WS_ADDR0_3.ipt
- C:\Users\caleb\Desktop\Shared\Software\Hardware\ETL\modules\Tamale v2.0\module_r50\WS_ADDR1.ipt
- C:\Users\caleb\Desktop\Shared\Software\Hardware\ETL\modules\Tamale v2.0\module_r50\WS_ADDR1_1.ipt
- C:\Users\caleb\Desktop\Shared\Software\Hardware\ETL\modules\Tamale v2.0\module_r50\WS_ADDR1_2.ipt
- C:\Users\caleb\Desktop\Shared\Software\Hardware\ETL\modules\Tamale v2.0\module_r50\WS_ADDR1_3.ipt
- C:\Users\caleb\Desktop\Shared\Software\Hardware\ETL\modules\Tamale v2.0\module_r50\WS_ADDR2.ipt
- C:\Users\caleb\Desktop\Shared\Software\Hardware\ETL\modules\Tamale v2.0\module_r50\WS_ADDR2_1.ipt
- C:\Users\caleb\Desktop\Shared\Software\Hardware\ETL\modules\Tamale v2.0\module_r50\WS_ADDR2_2.ipt
- C:\Users\caleb\Desktop\Shared\Software\Hardware\ETL\modules\Tamale v2.0\module_r50\WS_ADDR2_3.ipt
- C:\Users\caleb\Desktop\Shared\Software\Hardware\ETL\modules\Tamale v2.0\module_r50\WS_ADDR3.ipt
- C:\Users\caleb\Desktop\Shared\Software\Hardware\ETL\modules\Tamale v2.0\module_r50\WS_ADDR3_1.ipt
- C:\Users\caleb\Desktop\Shared\Software\Hardware\ETL\modules\Tamale v2.0\module_r50\WS_ADDR3_2.ipt
- C:\Users\caleb\Desktop\Shared\Software\Hardware\ETL\modules\Tamale v2.0\module_r50\WS_ADDR3_3.ipt
- C:\Users\caleb\Desktop\Shared\Software\Hardware\ETL\modules\Tamale v2.0\module_r50\WS_ADDR4.ipt
- C:\Users\caleb\Desktop\Shared\Software\Hardware\ETL\modules\Tamale v2.0\module_r50\WS_ADDR4_1.ipt
- C:\Users\caleb\Desktop\Shared\Software\Hardware\ETL\modules\Tamale v2.0\module_r50\WS_ADDR4_2.ipt
- C:\Users\caleb\Desktop\Shared\Software\Hardware\ETL\modules\Tamale v2.0\module_r50\WS_ADDR4_3.ipt
- C:\Users\caleb\Desktop\Shared\Software\Hardware\ETL\modules\Tamale v2.0\module_r50\WS_AVDD.ipt
- C:\Users\caleb\Desktop\Shared\Software\Hardware\ETL\modules\Tamale v2.0\module_r50\WS_AVDD_1.ipt
- C:\Users\caleb\Desktop\Shared\Software\Hardware\ETL\modules\Tamale v2.0\module_r50\WS_AVDD_2.ipt
- C:\Users\caleb\Desktop\Shared\Software\Hardware\ETL\modules\Tamale v2.0\module_r50\WS_AVDD_3.ipt
- C:\Users\caleb\Desktop\Shared\Software\Hardware\ETL\modules\Tamale v2.0\module_r50\WS_AVDD7.ipt
- C:\Users\caleb\Desktop\Shared\Software\Hardware\ETL\modules\Tamale v2.0\module_r50\WS_AVDD7_1.ipt
- C:\Users\caleb\Desktop\Shared\Software\Hardware\ETL\modules\Tamale v2.0\module_r50\WS_AVDD7_2.ipt
- C:\Users\caleb\Desktop\Shared\Software\Hardware\ETL\modules\Tamale v2.0\module_r50\WS_AVDD7_3.ipt